# Autodesk Inventor assembly: right_grabber
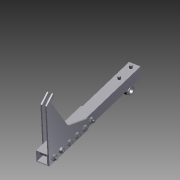
[picture p0: Inventor's stored thumbnail of the model, 180x180]
Saved by Autodesk Inventor 2011 (Build 150239000, 239)
## iProperties
Created: 2013-01-18
Part Number: right_grabber
Document SubType Name: Assembly
Designer: Christopher
Author: Christopher
## Documents named in this file (8)
- F:\Users\Christopher\Documents\GitHub\2013CAD\2013 robot\forklift\Pneumatics and frame grabbers\right_grabber.iam
- F:\Users\Christopher\Documents\GitHub\2013CAD\2013 robot\forklift\Pneumatics and frame grabbers\1tube_10_framegrabberarm.ipt
- F:\Users\Christopher\Documents\GitHub\2013CAD\2013 robot\forklift\Pneumatics and frame grabbers\grabber_plate_metal_hook.ipt
- F:\Users\Christopher\Documents\GitHub\2013CAD\2013 robot\forklift\Pneumatics and frame grabbers\grabber_plate_metal_hook_long.ipt
- F:\Users\Christopher\Documents\GitHub\2013CAD\2013 robot\forklift\Misc parts\1.5_bolt_.25_20.ipt
- F:\Users\Christopher\Documents\GitHub\2013CAD\2013 robot\forklift\Misc parts\nut_.25_20.ipt
- F:\Users\Christopher\Documents\GitHub\2013CAD\2013 robot\forklift\Misc parts\.5inch_side_bearing.ipt
- F:\Users\Christopher\Documents\GitHub\2013CAD\2013 robot\forklift\Misc parts\.5_inch_axle_bushing.ipt
## Components (20 placed, 7 different names)
1. 1tube_10_framegrabberarm:1 — Insert:3, Insert:4, Insert:21, Insert:22, Insert:23, Insert:24, Insert:25, Insert:26
2. grabber_plate_metal_hook:1 — Insert:5, Insert:6, Insert:7, Insert:8, Insert:9, Insert:23, Insert:24
3. grabber_plate_metal_hook_long:1 — Insert:3, Insert:4, Insert:10, Insert:11, Insert:12, Insert:13, Insert:14
4. 1.5_bolt_.25_20:1 — Insert:5
5. 1.5_bolt_.25_20:2 — Insert:6
6. 1.5_bolt_.25_20:3 — Insert:7
7. 1.5_bolt_.25_20:4 — Insert:8
8. 1.5_bolt_.25_20:5 — Insert:9
9. 1.5_bolt_.25_20:6 — Insert:20
10. 1.5_bolt_.25_20:7 — Insert:19
11. nut_.25_20:1 — Insert:10
12. nut_.25_20:2 — Insert:13
13. nut_.25_20:3 — Insert:14
14. nut_.25_20:4 — Insert:12
15. nut_.25_20:5 — Insert:11
16. .5inch_side_bearing:1 — Insert:17, Insert:18, Insert:19, Insert:20, Insert:21, Insert:22
17. .5_inch_axle_bushing:1 — Insert:17
18. .5_inch_axle_bushing:2 — Insert:18
19. 1.5_bolt_.25_20:8 — Insert:25
20. nut_.25_20:6 — Insert:26
## Relationships (22: Insert 22)
- Insert:3: 1tube_10_framegrabberarm:1 ↔ grabber_plate_metal_hook_long:1
- Insert:4: 1tube_10_framegrabberarm:1 ↔ grabber_plate_metal_hook_long:1
- Insert:5: grabber_plate_metal_hook:1 ↔ 1.5_bolt_.25_20:1
- Insert:6: grabber_plate_metal_hook:1 ↔ 1.5_bolt_.25_20:2
- Insert:7: grabber_plate_metal_hook:1 ↔ 1.5_bolt_.25_20:3
- Insert:8: grabber_plate_metal_hook:1 ↔ 1.5_bolt_.25_20:4
- Insert:9: grabber_plate_metal_hook:1 ↔ 1.5_bolt_.25_20:5
- Insert:10: grabber_plate_metal_hook_long:1 ↔ nut_.25_20:1
- Insert:11: grabber_plate_metal_hook_long:1 ↔ nut_.25_20:5
- Insert:12: grabber_plate_metal_hook_long:1 ↔ nut_.25_20:4
- Insert:13: grabber_plate_metal_hook_long:1 ↔ nut_.25_20:2
- Insert:14: grabber_plate_metal_hook_long:1 ↔ nut_.25_20:3
- Insert:17: .5inch_side_bearing:1 ↔ .5_inch_axle_bushing:1
- Insert:18: .5inch_side_bearing:1 ↔ .5_inch_axle_bushing:2
- Insert:19: 1.5_bolt_.25_20:7 ↔ .5inch_side_bearing:1
- Insert:20: 1.5_bolt_.25_20:6 ↔ .5inch_side_bearing:1
- Insert:21: 1tube_10_framegrabberarm:1 ↔ .5inch_side_bearing:1
- Insert:22: 1tube_10_framegrabberarm:1 ↔ .5inch_side_bearing:1
- Insert:23: 1tube_10_framegrabberarm:1 ↔ grabber_plate_metal_hook:1
- Insert:24: 1tube_10_framegrabberarm:1 ↔ grabber_plate_metal_hook:1
- Insert:25: 1tube_10_framegrabberarm:1 ↔ 1.5_bolt_.25_20:8
- Insert:26: 1tube_10_framegrabberarm:1 ↔ nut_.25_20:6
